# Autodesk Inventor assembly: SpeleoFox_front
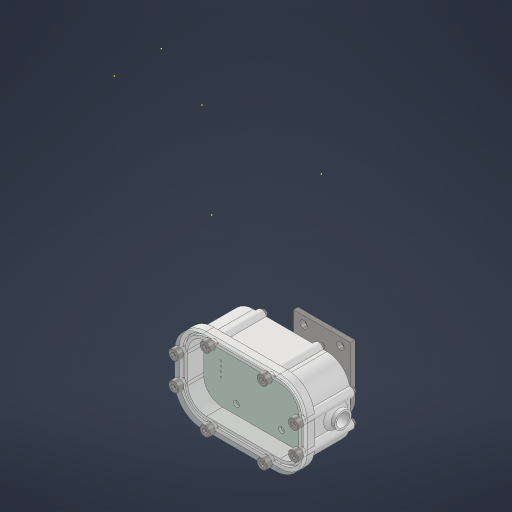
[picture p0: Inventor's stored thumbnail of the model, 512x512]
Saved by Autodesk Inventor 2024 (Build 280153000, 153)
## iProperties
Created: 2026-08-19
Part Number: SpeleoFox_front
Document SubType Name: Assembly
Designer: schar
Author: schar
## Documents named in this file (7)
- C:\Users\schar\Projects\SpeleoFox\cad\speleofox_parts\SpeleoFox_front.iam
- C:\Users\schar\Projects\SpeleoFox\cad\speleofox_parts\LED_speleopcb_part.ipt
- C:\Users\schar\Projects\SpeleoFox\cad\speleofox_parts\front_main_body.ipt
- C:\Users\schar\Projects\SpeleoFox\cad\speleofox_parts\front_acryl.ipt
- C:\Users\schar\Documents\Inventor\Content Center Files\R2024\en-US\DIN 912\DIN 912 - M3 x 0,5 x 30 x 18.ipt
- C:\Users\schar\Projects\SpeleoFox\cad\speleofox_parts\helmet_holder.ipt
- C:\Users\schar\Projects\SpeleoFox\cad\speleofox_parts\AST13SEBQ.ipt
## Components (13 placed, 6 different names)
1. LED_speleopcb_part:1 — Flush:1, Flush:2
2. front_main_body:1 — Flush:1, Flush:2, Flush:3, Mate:2, Flush:4, Flush:5, Flush:6
3. front_acryl:1 — Flush:3, Mate:1, Mate:3, Mate:4, Mate:5, Mate:6, Mate:7, Mate:8, Mate:9, Mate:10, Mate:11, Mate:12, Mate:13, Mate:14, Mate:15, Mate:16
4. DIN 912 - replaced by DIN EN ISO 4762 M3 x 30:1 — Mate:1, Mate:2
5. DIN 912 - replaced by DIN EN ISO 4762 M3 x 30:2 — Mate:3, Mate:6
6. DIN 912 - replaced by DIN EN ISO 4762 M3 x 30:3 — Mate:4, Mate:5
7. helmet_holder:1 — Flush:4
8. AST13SEBQ:1 — Flush:5, Flush:6
9. DIN 912 - replaced by DIN EN ISO 4762 M3 x 30:4 — Mate:7, Mate:16
10. DIN 912 - replaced by DIN EN ISO 4762 M3 x 30:5 — Mate:8, Mate:15
11. DIN 912 - replaced by DIN EN ISO 4762 M3 x 30:6 — Mate:9, Mate:14
12. DIN 912 - replaced by DIN EN ISO 4762 M3 x 30:7 — Mate:10, Mate:13
13. DIN 912 - replaced by DIN EN ISO 4762 M3 x 30:8 — Mate:11, Mate:12
## Relationships (22: Mate 16, Flush 6)
- Flush:1: LED_speleopcb_part:1 ↔ front_main_body:1
- Flush:2: LED_speleopcb_part:1 ↔ front_main_body:1
- Flush:3: front_main_body:1 ↔ front_acryl:1
- Mate:1: front_acryl:1 ↔ DIN 912 - replaced by DIN EN ISO 4762 M3 x 30:1
- Mate:2: front_main_body:1 ↔ DIN 912 - replaced by DIN EN ISO 4762 M3 x 30:1
- Mate:3: front_acryl:1 ↔ DIN 912 - replaced by DIN EN ISO 4762 M3 x 30:2
- Mate:4: front_acryl:1 ↔ DIN 912 - replaced by DIN EN ISO 4762 M3 x 30:3
- Mate:5: front_acryl:1 ↔ DIN 912 - replaced by DIN EN ISO 4762 M3 x 30:3
- Mate:6: front_acryl:1 ↔ DIN 912 - replaced by DIN EN ISO 4762 M3 x 30:2
- Flush:4: front_main_body:1 ↔ helmet_holder:1
- Flush:5: front_main_body:1 ↔ AST13SEBQ:1
- Flush:6: front_main_body:1 ↔ AST13SEBQ:1
- Mate:7: front_acryl:1 ↔ DIN 912 - replaced by DIN EN ISO 4762 M3 x 30:4
- Mate:8: front_acryl:1 ↔ DIN 912 - replaced by DIN EN ISO 4762 M3 x 30:5
- Mate:9: front_acryl:1 ↔ DIN 912 - replaced by DIN EN ISO 4762 M3 x 30:6
- Mate:10: front_acryl:1 ↔ DIN 912 - replaced by DIN EN ISO 4762 M3 x 30:7
- Mate:11: front_acryl:1 ↔ DIN 912 - replaced by DIN EN ISO 4762 M3 x 30:8
- Mate:12: front_acryl:1 ↔ DIN 912 - replaced by DIN EN ISO 4762 M3 x 30:8
- Mate:13: front_acryl:1 ↔ DIN 912 - replaced by DIN EN ISO 4762 M3 x 30:7
- Mate:14: front_acryl:1 ↔ DIN 912 - replaced by DIN EN ISO 4762 M3 x 30:6
- Mate:15: front_acryl:1 ↔ DIN 912 - replaced by DIN EN ISO 4762 M3 x 30:5
- Mate:16: front_acryl:1 ↔ DIN 912 - replaced by DIN EN ISO 4762 M3 x 30:4
